# Autodesk Inventor assembly: CHA_000_Chassis
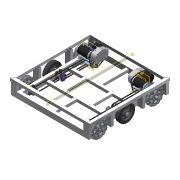
[picture p0: Inventor's stored thumbnail of the model, 180x180]
Saved by Autodesk Inventor 2020 (Build 240168000, 168)
## iProperties
Created: 2020-01-10
Part Number: CHA_000_Chassis
Document SubType Name: Assembly
Designer: user
Mass: 13129.8 g
Surface Area: 43463.5 cm^2
Volume: 8744.12 cm^3
Density: 1.50156 g/cm^3
Author: user
## Documents named in this file (21)
- C:\Users\mdill\Documents\GrabCAD\Infinite Recharge 2020\Build season\CHA_000_FullChassis.iam
- C:\Users\mdill\Documents\GrabCAD\Infinite Recharge 2020\Build season\FRA_000_FullFrame.iam
- C:\Users\mdill\Documents\GrabCAD\Infinite Recharge 2020\Build season\VersaBlock_V2_217-6111_Combined.iam
- C:\Users\mdill\Documents\GrabCAD\Infinite Recharge 2020\Build season\WCP_Gearbox_Bearing_Block_217-3634.ipt
- C:\Users\mdill\Documents\GrabCAD\Infinite Recharge 2020\Build season\DGB_000_DriveGearBox.iam
- C:\Users\mdill\Documents\GrabCAD\Infinite Recharge 2020\Brainstorming\The Hooded Shooter\6In Fly Hooded Shooter\WH_Colsons6_000.iam
- C:\Users\mdill\Documents\GrabCAD\Infinite Recharge 2020\Build season\DGB STEP\217-2731_0_500_flanged_bearing.ipt
- C:\Users\mdill\Documents\GrabCAD\Infinite Recharge 2020\Build season\CHA_001_CenterDriveAxle.ipt
- C:\Users\mdill\Documents\GrabCAD\Infinite Recharge 2020\Build season\CHA_002_FarDriveAxle.ipt
- C:\Users\mdill\Documents\GrabCAD\Infinite Recharge 2020\Build season\OMNIWHEEL STEP\6_Omni-Directional_Wheel_217-2585.iam
- C:\Users\mdill\Documents\GrabCAD\Infinite Recharge 2020\Build season\CHA_007_DrivenPulleyAssembly.iam
- C:\Users\mdill\Documents\GrabCAD\Infinite Recharge 2020\Build season\CHA_009_AngleHexBolt.ipt
- C:\Users\mdill\Documents\GrabCAD\Infinite Recharge 2020\Build season\VersaBlock_V2_217-6111_Combined_MIR.iam
- C:\Users\mdill\Documents\GrabCAD\Infinite Recharge 2020\Build season\CHA_001_CenterDriveAxle_MIR.ipt
- C:\Users\mdill\Documents\GrabCAD\Infinite Recharge 2020\Build season\CHA_002_FarDriveAxle_MIR.ipt
- C:\Users\mdill\Documents\GrabCAD\Infinite Recharge 2020\Build season\CHA_007_DrivenPulleyAssembly_MIR.iam
- C:\Users\mdill\Documents\GrabCAD\Infinite Recharge 2020\Build season\WCP_Gearbox_Bearing_Block_217-3634_MIR.ipt
- C:\Users\mdill\Documents\GrabCAD\Infinite Recharge 2020\Build season\DGB STEP\217-2731_0_500_flanged_bearing_MIR1.ipt
- C:\Users\mdill\Documents\GrabCAD\Infinite Recharge 2020\Build season\DGB_005_Short Belt_Gates_695-5M-09.ipt
- C:\Users\mdill\Documents\GrabCAD\Infinite Recharge 2020\Build season\DGB_006_LonG Belt_Gates_1200-5M-09.ipt
- C:\Users\mdill\Documents\GrabCAD\Infinite Recharge 2020\Build season\DGB_000_DriveGearBox_MIR3.iam
## Components (33 placed, 20 different names)
1. FRA_000_FullFrame:1 [sub-assembly] — Mate:2, Mate:4, Mate:5, Flush:1, Insert:1, Mate:6, Mate:8, Angle:2, Insert:3, Insert:4, Mate:89, Mate:90, Mate:91, Mate:92, Mate:101, Insert:6, Insert:7, Mate:7, Angle:3, Angle:4
2. VersaBlock_V2_217-6111_Combined:1 [sub-assembly] — Mate:4, Flush:1, Mate:14, Mate:104
3. VersaBlock_V2_217-6111_Combined:2 [sub-assembly] — Mate:2, Mate:5, Mate:15, Mate:140
4. WCP_Gearbox_Bearing_Block_217-3634:1 — Insert:1, Mate:6, Insert:2, Mate:127, Mate:143
5. DGB_000_DriveGearBox:1 [sub-assembly] — Mate:7, Mate:127, Angle:3, Mate:141, Mate:142
6. 217-2731_0_500_flanged_bearing:1 — Insert:2
7. CHA_001_CenterDriveAxle:1 — Mate:15, Mate:22, Mate:23, Flush:5, Mate:128, Flush:16, Mate:129
8. CHA_002_FarDriveAxle:1 — Mate:14, Mate:24, Mate:25, Flush:4, Mate:102, Mate:103
9. CHA_007_DrivenPulleyAssembly:1 [sub-assembly] — Mate:24, Mate:25, Flush:4, Mate:139
10. CHA_007_DrivenPulleyAssembly:2 [sub-assembly] — Mate:22, Mate:23, Flush:5, Mate:138
11. WH_Colsons6_000:2 [sub-assembly] — Mate:128, Flush:16, Mate:129, Mate:140
12. Hex Bolt - Inch 1/4-20 UNC - 5:1 — Insert:4
13. Hex Bolt - Inch 1/4-20 UNC - 5:2 — Insert:3
14. VersaBlock_V2_217-6111_Combined_MIR:1 [sub-assembly] — Mate:70, Mate:91, Mate:92
15. VersaBlock_V2_217-6111_Combined_MIR:2 [sub-assembly] — Mate:69, Mate:89, Mate:90
16. CHA_001_CenterDriveAxle_MIR:1 — Mate:69, Flush:12, Mate:73, Mate:74, Mate:130, Flush:17, Mate:131
17. CHA_002_FarDriveAxle_MIR:1 — Mate:70, Flush:10, Mate:71, Mate:72, Mate:99, Mate:100
18. CHA_007_DrivenPulleyAssembly_MIR:1 [sub-assembly] — Flush:10, Mate:71, Mate:72, Mate:137
19. CHA_007_DrivenPulleyAssembly_MIR:2 [sub-assembly] — Flush:12, Mate:73, Mate:74, Mate:136
20. WH_Colsons6_000:3 [sub-assembly] — Mate:130, Flush:17, Mate:131
21. WCP_Gearbox_Bearing_Block_217-3634_MIR:1 — Insert:5, Mate:146
22. 217-2731_0_500_flanged_bearing_MIR1:1 — Insert:5
23. Hex Bolt - Inch 1/4-20 UNC - 5:3 — Insert:6
24. Hex Bolt - Inch 1/4-20 UNC - 5:4 — Insert:7
25. 6_Omni-Directional_Wheel_217-2585:2 [sub-assembly] — Mate:99, Mate:100, Mate:101
26. 6_Omni-Directional_Wheel_217-2585:3 [sub-assembly] — Mate:102, Mate:103, Mate:104
27. DGB_005_Short Belt_Gates_695-5M-09:1 — Mate:132, Flush:19, Flush:20, Flush:21, Mate:138
28. DGB_005_Short Belt_Gates_695-5M-09:2 — Mate:132, Mate:133, Mate:134, Flush:21, Angle:4, Mate:136
29. DGB_006_LonG Belt_Gates_1200-5M-09:1 — Mate:133, Flush:19, Mate:139
30. DGB_006_LonG Belt_Gates_1200-5M-09:2 — Mate:134, Flush:20, Mate:137
31. 6_Omni-Directional_Wheel_217-2585:4 [sub-assembly] — Mate:146
32. 6_Omni-Directional_Wheel_217-2585:5 [sub-assembly] — Mate:141, Mate:142, Mate:143
33. DGB_000_DriveGearBox_MIR3:1 [sub-assembly]
## Relationships (66: Mate 45, Flush 11, Insert 7, Angle 3)
- Mate:2: FRA_000_FullFrame:1 ↔ VersaBlock_V2_217-6111_Combined:2
- Mate:4: FRA_000_FullFrame:1 ↔ VersaBlock_V2_217-6111_Combined:1
- Mate:5: FRA_000_FullFrame:1 ↔ VersaBlock_V2_217-6111_Combined:2
- Flush:1: FRA_000_FullFrame:1 ↔ VersaBlock_V2_217-6111_Combined:1
- Insert:1: FRA_000_FullFrame:1 ↔ WCP_Gearbox_Bearing_Block_217-3634:1
- Mate:6: FRA_000_FullFrame:1 ↔ WCP_Gearbox_Bearing_Block_217-3634:1
- Mate:7: FRA_000_FullFrame:1 ↔ DGB_000_DriveGearBox:1
- Mate:8: FRA_000_FullFrame:1
- Angle:2 (0 deg): FRA_000_FullFrame:1
- Insert:2: WCP_Gearbox_Bearing_Block_217-3634:1 ↔ 217-2731_0_500_flanged_bearing:1
- Mate:14: VersaBlock_V2_217-6111_Combined:1 ↔ CHA_002_FarDriveAxle:1
- Mate:15: VersaBlock_V2_217-6111_Combined:2 ↔ CHA_001_CenterDriveAxle:1
- Mate:22: CHA_001_CenterDriveAxle:1 ↔ CHA_007_DrivenPulleyAssembly:2
- Mate:23: CHA_001_CenterDriveAxle:1 ↔ CHA_007_DrivenPulleyAssembly:2
- Mate:24: CHA_002_FarDriveAxle:1 ↔ CHA_007_DrivenPulleyAssembly:1
- Mate:25: CHA_002_FarDriveAxle:1 ↔ CHA_007_DrivenPulleyAssembly:1
- Flush:4: CHA_002_FarDriveAxle:1 ↔ CHA_007_DrivenPulleyAssembly:1
- Flush:5: CHA_001_CenterDriveAxle:1 ↔ CHA_007_DrivenPulleyAssembly:2
- Insert:3: FRA_000_FullFrame:1 ↔ Hex Bolt - Inch 1/4-20 UNC - 5:2
- Insert:4: FRA_000_FullFrame:1 ↔ Hex Bolt - Inch 1/4-20 UNC - 5:1
- Mate:69: VersaBlock_V2_217-6111_Combined_MIR:2 ↔ CHA_001_CenterDriveAxle_MIR:1
- Mate:70: VersaBlock_V2_217-6111_Combined_MIR:1 ↔ CHA_002_FarDriveAxle_MIR:1
- Flush:10: CHA_002_FarDriveAxle_MIR:1 ↔ CHA_007_DrivenPulleyAssembly_MIR:1
- Mate:71: CHA_002_FarDriveAxle_MIR:1 ↔ CHA_007_DrivenPulleyAssembly_MIR:1
- Mate:72: CHA_002_FarDriveAxle_MIR:1 ↔ CHA_007_DrivenPulleyAssembly_MIR:1
- Flush:12: CHA_001_CenterDriveAxle_MIR:1 ↔ CHA_007_DrivenPulleyAssembly_MIR:2
- Mate:73: CHA_001_CenterDriveAxle_MIR:1 ↔ CHA_007_DrivenPulleyAssembly_MIR:2
- Mate:74: CHA_001_CenterDriveAxle_MIR:1 ↔ CHA_007_DrivenPulleyAssembly_MIR:2
- Insert:5: WCP_Gearbox_Bearing_Block_217-3634_MIR:1 ↔ 217-2731_0_500_flanged_bearing_MIR1:1
- Mate:89: FRA_000_FullFrame:1 ↔ VersaBlock_V2_217-6111_Combined_MIR:2
- Mate:90: FRA_000_FullFrame:1 ↔ VersaBlock_V2_217-6111_Combined_MIR:2
- Mate:91: FRA_000_FullFrame:1 ↔ VersaBlock_V2_217-6111_Combined_MIR:1
- Mate:92: FRA_000_FullFrame:1 ↔ VersaBlock_V2_217-6111_Combined_MIR:1
- Mate:99: CHA_002_FarDriveAxle_MIR:1 ↔ 6_Omni-Directional_Wheel_217-2585:2
- Mate:100: CHA_002_FarDriveAxle_MIR:1 ↔ 6_Omni-Directional_Wheel_217-2585:2
- Mate:101 (7.5692 mm): FRA_000_FullFrame:1 ↔ 6_Omni-Directional_Wheel_217-2585:2
- Mate:102: CHA_002_FarDriveAxle:1 ↔ 6_Omni-Directional_Wheel_217-2585:3
- Mate:103: CHA_002_FarDriveAxle:1 ↔ 6_Omni-Directional_Wheel_217-2585:3
- Mate:104 (7.5692 mm): VersaBlock_V2_217-6111_Combined:1 ↔ 6_Omni-Directional_Wheel_217-2585:3
- Insert:6: FRA_000_FullFrame:1 ↔ Hex Bolt - Inch 1/4-20 UNC - 5:3
- Insert:7: FRA_000_FullFrame:1 ↔ Hex Bolt - Inch 1/4-20 UNC - 5:4
- Flush:15 (-69.85 mm)
- Mate:127: WCP_Gearbox_Bearing_Block_217-3634:1 ↔ DGB_000_DriveGearBox:1
- Angle:3 (180 deg): FRA_000_FullFrame:1 ↔ DGB_000_DriveGearBox:1
- Mate:128: CHA_001_CenterDriveAxle:1 ↔ WH_Colsons6_000:2
- Flush:16: CHA_001_CenterDriveAxle:1 ↔ WH_Colsons6_000:2
- Mate:129: CHA_001_CenterDriveAxle:1 ↔ WH_Colsons6_000:2
- Mate:130: CHA_001_CenterDriveAxle_MIR:1 ↔ WH_Colsons6_000:3
- Flush:17: CHA_001_CenterDriveAxle_MIR:1 ↔ WH_Colsons6_000:3
- Mate:131: CHA_001_CenterDriveAxle_MIR:1 ↔ WH_Colsons6_000:3
- Mate:132: DGB_005_Short Belt_Gates_695-5M-09:1 ↔ DGB_005_Short Belt_Gates_695-5M-09:2
- Mate:133: DGB_005_Short Belt_Gates_695-5M-09:2 ↔ DGB_006_LonG Belt_Gates_1200-5M-09:1
- Mate:134: DGB_005_Short Belt_Gates_695-5M-09:2 ↔ DGB_006_LonG Belt_Gates_1200-5M-09:2
- Flush:19: DGB_005_Short Belt_Gates_695-5M-09:1 ↔ DGB_006_LonG Belt_Gates_1200-5M-09:1
- Flush:20: DGB_005_Short Belt_Gates_695-5M-09:1 ↔ DGB_006_LonG Belt_Gates_1200-5M-09:2
- Flush:21: DGB_005_Short Belt_Gates_695-5M-09:1 ↔ DGB_005_Short Belt_Gates_695-5M-09:2
- Angle:4 (0 deg): FRA_000_FullFrame:1 ↔ DGB_005_Short Belt_Gates_695-5M-09:2
- Mate:136 (3.7427 mm): CHA_007_DrivenPulleyAssembly_MIR:2 ↔ DGB_005_Short Belt_Gates_695-5M-09:2
- Mate:137 (3.7427 mm): CHA_007_DrivenPulleyAssembly_MIR:1 ↔ DGB_006_LonG Belt_Gates_1200-5M-09:2
- Mate:138 (3.7427 mm): CHA_007_DrivenPulleyAssembly:2 ↔ DGB_005_Short Belt_Gates_695-5M-09:1
- Mate:139 (3.7427 mm): CHA_007_DrivenPulleyAssembly:1 ↔ DGB_006_LonG Belt_Gates_1200-5M-09:1
- Mate:140: VersaBlock_V2_217-6111_Combined:2 ↔ WH_Colsons6_000:2
- Mate:141: DGB_000_DriveGearBox:1 ↔ 6_Omni-Directional_Wheel_217-2585:5
- Mate:142: DGB_000_DriveGearBox:1 ↔ 6_Omni-Directional_Wheel_217-2585:5
- Mate:143 (7.5692 mm): WCP_Gearbox_Bearing_Block_217-3634:1 ↔ 6_Omni-Directional_Wheel_217-2585:5
- Mate:146: WCP_Gearbox_Bearing_Block_217-3634_MIR:1 ↔ 6_Omni-Directional_Wheel_217-2585:4
